# Autodesk Inventor assembly: Ensamble-Efector final
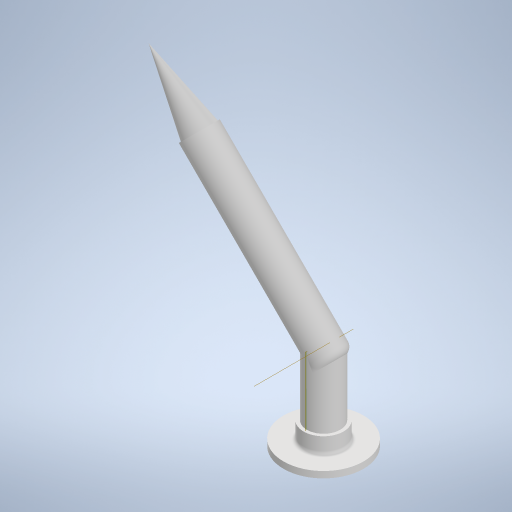
[picture p0: Inventor's stored thumbnail of the model, 512x512]
Saved by Autodesk Inventor 2023 (Build 270158000, 158)
## iProperties
Created: 2024-03-01
Part Number: Ensamble-Efector final
Document SubType Name: Assembly
Designer: LENOVO
Author: LENOVO
## Documents named in this file (3)
- C:\Users\LENOVO\Desktop\UN\Décimo semestre\Robótica\Laboratorios\Laboratorio 1\Ensamble-Efector final.iam
- C:\Users\LENOVO\Desktop\UN\Décimo semestre\Robótica\Laboratorios\Laboratorio 1\Brida.ipt
- C:\Users\LENOVO\Desktop\UN\Décimo semestre\Robótica\Laboratorios\Laboratorio 1\Efector final.ipt
## Components (2 placed, 2 different names)
1. Brida:1 — Rigid:1
2. Efector final:1 — Rigid:1
## Relationships (1: WeldJoint 1)
- Rigid:1 [WeldJoint]: Brida:1 ↔ Efector final:1
